# Autodesk Inventor assembly: OBG-Antrieb Getriebe
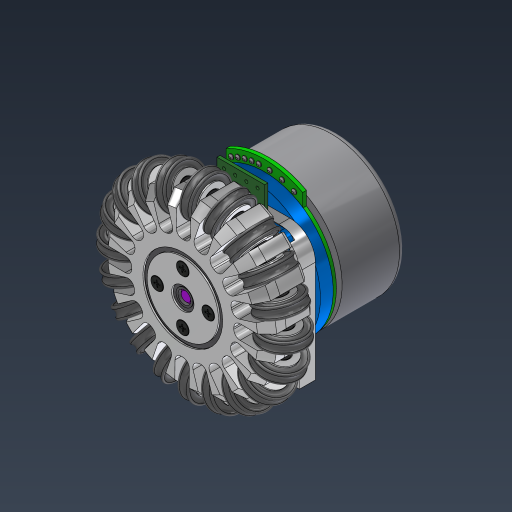
[picture p0: Inventor's stored thumbnail of the model, 512x512]
Saved by Autodesk Inventor 2023.1 (Build 271208000, 208)
## iProperties
Part Number: OBG-Antrieb Getriebe
Material: Generisch
Document SubType Name: Assembly
Designer: rYan
Mass: 234.467 g
Surface Area: 734.726 cm^2
Volume: 67.3795 cm^3
Density: 3.4798 g/cm^3
Author: rYan
## Documents named in this file (18)
- D:\TIGERsGIT\Hardware\mechanik\2024\Inventor\Robot\Drive Train\Geared\OBG-Antrieb Getriebe.iam
- D:\TIGERsGIT\Hardware\mechanik\2024\Inventor\Robot\Drive Train\Geared\Lagerbock Getriebe.ipt
- D:\TIGERsGIT\Hardware\mechanik\2024\Inventor\Purchased Parts\DF45L024048\DF45L024048-A2.iam
- D:\TIGERsGIT\Hardware\mechanik\2024\Inventor\Robot\Drive Train\Geared\UBG-Rad Getriebe.iam
- D:\TIGERsGIT\Hardware\mechanik\2024\Inventor\Robot\Drive Train\Common\MG-Encoderplatine.iam
- D:\TIGERsGIT\Hardware\mechanik\2024\Inventor\Purchased Parts\iC-Haus PX01S 26-360.ipt
- D:\TIGERsGIT\Hardware\mechanik\2024\Inventor\Robot\Drive Train\Geared\Encoder Disk Halter.ipt
- D:\TIGERsGIT\Hardware\mechanik\2024\Inventor\Robot\Drive Train\Geared\Getriebe Planetenhalter.ipt
- D:\TIGERsGIT\Hardware\mechanik\2024\Inventor\Robot\Drive Train\Geared\Encoder Klemmscheibe.ipt
- D:\TIGERsGIT\Hardware\mechanik\2024\Inventor\Inhaltscenter\de-DE\ISO 7046-1 H(1)\ISO 7046-1 - M2 x 4_ - 4.8 - H - ISO.ipt
- D:\TIGERsGIT\Hardware\mechanik\2024\Inventor\Inhaltscenter\de-DE\DIN 7984\DIN 7984 - M3 x 5.ipt
- D:\TIGERsGIT\Hardware\mechanik\2024\Inventor\Purchased Parts\ISO 10642 - M3 x 4.ipt
- D:\TIGERsGIT\Hardware\mechanik\2024\Inventor\Robot\Drive Train\Geared\Planetengetriebe Planet.ipt
- D:\TIGERsGIT\Hardware\mechanik\2024\Inventor\Robot\Drive Train\Geared\Planetengetriebe Sonne.ipt
- D:\TIGERsGIT\Hardware\mechanik\2024\Inventor\Inhaltscenter\de-DE\ISO 7046-1 H(1)\ISO 7046-1 - M2 x 10_ - 4.8 - H - ISO.ipt
- D:\TIGERsGIT\Hardware\mechanik\2024\Inventor\Robot\Drive Train\Geared\Getriebe Abdeckung.ipt
- D:\TIGERsGIT\Hardware\mechanik\2024\Inventor\Purchased Parts\Kugellager 684-2RS.ipt
- D:\TIGERsGIT\Hardware\mechanik\2024\Inventor\Inhaltscenter\de-DE\ISO 4762(1)\DIN EN ISO 4762 - M2 x 4.ipt
## Components (29 placed, 17 different names)
1. Lagerbock:1 — Passend:26, Passend:68, Passend:69, Einfügen:5, Passend:70, Einfügen:9, Winkel:1, Winkel:2, Einfügen:37, Einfügen:38, Einfügen:39, Nullpos Sonne, Winkel:4, Winkel:5
2. DF45L024048-A2:1 [sub-assembly] — Passend:26, Passend:62, Passend:68, Passend:69, Einfügen:28, Passend:72
3. UBG-Rad:1 [sub-assembly] — Winkel:2, Einfügen:47, Einfügen:52, Drehung:5
4. MG-Encoderplatine:1 [sub-assembly] — Passend:63, Einfügen:5, Passend:70, Einfügen:35, Einfügen:40
5. iC-Haus PX01S 26-360:1 — Passend:62, Passend:63, Einfügen:56
6. Encoder Disk Halter:1 — Einfügen:56
7. Getriebe Planetenhalter:1 — Einfügen:9, Winkel:1, Einfügen:29, Einfügen:31, Einfügen:32, Einfügen:33, Einfügen:47, Einfügen:48, Einfügen:50, Passend:74
8. Encoder Klemmscheibe:1 — Einfügen:28, Einfügen:57, Winkel:79, Einfügen:58, Einfügen:59
9. Planetengetriebe Sonne z7:1 — Passend:72, Nullpos Sonne, Drehung:2, Drehung:4, Drehung:5, Winkel:79, Passend:75
10. Planetengetriebe Planet z9:2 — Einfügen:48, Winkel:4, Drehung:2
11. Planetengetriebe Planet z9:4 — Einfügen:50, Winkel:5, Drehung:4
12. Getriebe Abdeckung:1 — Einfügen:51, Einfügen:52, Einfügen:46, Passend:74, Einfügen:53, Einfügen:54, Einfügen:55
13. Kugellager 684-2RS:1 — Einfügen:51, Passend:75
14. ISO 10642 M3 x  4:5 — Einfügen:29
15. ISO 10642 M3 x  4:6 — Einfügen:31
16. ISO 10642 M3 x  4:7 — Einfügen:32
17. ISO 10642 M3 x  4:8 — Einfügen:33
18. ISO 7046-1 H M2 x 4 - 4.8 - H:1 — Einfügen:35
19. DIN 7984 M3 x 5:1 — Einfügen:37
20. DIN 7984 M3 x 5:2 — Einfügen:38
21. DIN 7984 M3 x 5:3 — Einfügen:39
22. ISO 7046-1 H M2 x 4 - 4.8 - H:2 — Einfügen:40
23. ISO 7046-1 H M2 x 10 - 4.8 - H:1 — Einfügen:46
24. ISO 7046-1 H M2 x 10 - 4.8 - H:2 — Einfügen:53
25. ISO 7046-1 H M2 x 10 - 4.8 - H:3 — Einfügen:54
26. ISO 7046-1 H M2 x 10 - 4.8 - H:4 — Einfügen:55
27. DIN EN ISO 4762 M2 x 4:1 — Einfügen:57
28. DIN EN ISO 4762 M2 x 4:2 — Einfügen:58
29. DIN EN ISO 4762 M2 x 4:3 — Einfügen:59
## Relationships (43: Insert 25, Mate 9, Angle 5, RelateRotation 3, Flush 1)
- Passend:26 [Mate]: Lagerbock:1 ↔ DF45L024048-A2:1
- Passend:62 [Mate]: DF45L024048-A2:1 ↔ iC-Haus PX01S 26-360:1
- Passend:63 [Mate] (1.5 mm): MG-Encoderplatine:1 ↔ iC-Haus PX01S 26-360:1
- Passend:68 [Mate]: Lagerbock:1 ↔ DF45L024048-A2:1
- Passend:69 [Mate]: Lagerbock:1 ↔ DF45L024048-A2:1
- Einfügen:5 [Insert]: Lagerbock:1 ↔ MG-Encoderplatine:1
- Passend:70 [Mate]: Lagerbock:1 ↔ MG-Encoderplatine:1
- Einfügen:9 [Insert]: Lagerbock:1 ↔ Getriebe Planetenhalter:1
- Winkel:1 [Angle] (0 deg): Lagerbock:1 ↔ Getriebe Planetenhalter:1
- Winkel:2 [Angle] (0 deg): Lagerbock:1 ↔ UBG-Rad:1
- Einfügen:28 [Insert] (1 mm): DF45L024048-A2:1 ↔ Encoder Klemmscheibe:1
- Einfügen:29 [Insert] (-0.1 mm): Getriebe Planetenhalter:1 ↔ ISO 10642 M3 x  4:5
- Einfügen:31 [Insert] (-0.1 mm): Getriebe Planetenhalter:1 ↔ ISO 10642 M3 x  4:6
- Einfügen:32 [Insert] (-0.1 mm): Getriebe Planetenhalter:1 ↔ ISO 10642 M3 x  4:7
- Einfügen:33 [Insert] (-0.1 mm): Getriebe Planetenhalter:1 ↔ ISO 10642 M3 x  4:8
- Einfügen:35 [Insert] (-0.2 mm): MG-Encoderplatine:1 ↔ ISO 7046-1 H M2 x 4 - 4.8 - H:1
- Einfügen:37 [Insert]: Lagerbock:1 ↔ DIN 7984 M3 x 5:1
- Einfügen:38 [Insert]: Lagerbock:1 ↔ DIN 7984 M3 x 5:2
- Einfügen:39 [Insert]: Lagerbock:1 ↔ DIN 7984 M3 x 5:3
- Einfügen:40 [Insert] (-0.2 mm): MG-Encoderplatine:1 ↔ ISO 7046-1 H M2 x 4 - 4.8 - H:2
- Passend:72 [Mate]: DF45L024048-A2:1 ↔ Planetengetriebe Sonne z7:1
- Einfügen:46 [Insert] (-0.1 mm): Getriebe Abdeckung:1 ↔ ISO 7046-1 H M2 x 10 - 4.8 - H:1
- Einfügen:47 [Insert] (1.1 mm): UBG-Rad:1 ↔ Getriebe Planetenhalter:1
- Einfügen:48 [Insert]: Getriebe Planetenhalter:1 ↔ Planetengetriebe Planet z9:2
- Einfügen:50 [Insert]: Getriebe Planetenhalter:1 ↔ Planetengetriebe Planet z9:4
- Einfügen:51 [Insert]: Getriebe Abdeckung:1 ↔ Kugellager 684-2RS:1
- Einfügen:52 [Insert]: UBG-Rad:1 ↔ Getriebe Abdeckung:1
- Passend:74 [Mate]: Getriebe Planetenhalter:1 ↔ Getriebe Abdeckung:1
- Einfügen:53 [Insert] (-0.1 mm): Getriebe Abdeckung:1 ↔ ISO 7046-1 H M2 x 10 - 4.8 - H:2
- Einfügen:54 [Insert] (-0.1 mm): Getriebe Abdeckung:1 ↔ ISO 7046-1 H M2 x 10 - 4.8 - H:3
- Nullpos Sonne [Flush]: Lagerbock:1 ↔ Planetengetriebe Sonne z7:1
- Winkel:4 [Angle] (38.5 deg): Lagerbock:1 ↔ Planetengetriebe Planet z9:2
- Winkel:5 [Angle] (0 deg): Lagerbock:1 ↔ Planetengetriebe Planet z9:4
- Drehung:2 [RelateRotation] (1.2857 ul): Planetengetriebe Sonne z7:1 ↔ Planetengetriebe Planet z9:2
- Drehung:4 [RelateRotation] (1.2857 ul): Planetengetriebe Sonne z7:1 ↔ Planetengetriebe Planet z9:4
- Drehung:5 [RelateRotation] (0.3913 ul): UBG-Rad:1 ↔ Planetengetriebe Sonne z7:1
- Einfügen:55 [Insert] (-0.1 mm): Getriebe Abdeckung:1 ↔ ISO 7046-1 H M2 x 10 - 4.8 - H:4
- Einfügen:56 [Insert]: iC-Haus PX01S 26-360:1 ↔ Encoder Disk Halter:1
- Einfügen:57 [Insert] (0.15 mm): Encoder Klemmscheibe:1 ↔ DIN EN ISO 4762 M2 x 4:1
- Winkel:79 [Angle] (180 deg): Encoder Klemmscheibe:1 ↔ Planetengetriebe Sonne z7:1
- Passend:75 [Mate] (-0.95 mm): Planetengetriebe Sonne z7:1 ↔ Kugellager 684-2RS:1
- Einfügen:58 [Insert]: Encoder Klemmscheibe:1 ↔ DIN EN ISO 4762 M2 x 4:2
- Einfügen:59 [Insert]: Encoder Klemmscheibe:1 ↔ DIN EN ISO 4762 M2 x 4:3
